# Autodesk Inventor assembly: Assembly1
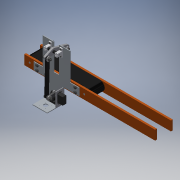
[picture p0: Inventor's stored thumbnail of the model, 180x180]
Saved by Autodesk Inventor 2019 (Build 230136000, 136)
## iProperties
Created: 2021-10-24
Part Number: Assembly1
Document SubType Name: Assembly
Designer: Mohamed Teleb
Sending System: Autodesk Inventor 2022
Preprocessor: ST-DEVELOPER v18.1
Title: C:\Users\Mohamed Teleb\OneDrive - Faculty of Engineering Ain Shams University\Documents\Inventor\AssemblyDesignOfMechatronics1\Assembly1.stp
Author: Mohamed Teleb
## Documents named in this file (32)
- C:\Users\Mohamed Teleb\OneDrive - Faculty of Engineering Ain Shams University\Desktop\DOM1STEP\Assembly1.iam
- C:\Users\Mohamed Teleb\OneDrive - Faculty of Engineering Ain Shams University\Desktop\DOM1STEP\Part1.ipt
- C:\Users\Mohamed Teleb\OneDrive - Faculty of Engineering Ain Shams University\Desktop\DOM1STEP\Part4.ipt
- C:\Users\Mohamed Teleb\OneDrive - Faculty of Engineering Ain Shams University\Desktop\DOM1STEP\Part7.ipt
- C:\Users\Mohamed Teleb\OneDrive - Faculty of Engineering Ain Shams University\Desktop\DOM1STEP\FilesFromInventor2019\SideToConveyer.ipt
- C:\Users\Mohamed Teleb\OneDrive - Faculty of Engineering Ain Shams University\Desktop\DOM1STEP\ISO 14583 - M8x25-4.8.ipt
- C:\Users\Mohamed Teleb\OneDrive - Faculty of Engineering Ain Shams University\Desktop\DOM1STEP\ISO 8738 - 8(2).ipt
- C:\Users\Mohamed Teleb\OneDrive - Faculty of Engineering Ain Shams University\Desktop\DOM1STEP\ISO 4034 - M8 - ISO.ipt
- C:\Users\Mohamed Teleb\OneDrive - Faculty of Engineering Ain Shams University\Desktop\DOM1STEP\StepperHolder.ipt
- C:\Users\Mohamed Teleb\OneDrive - Faculty of Engineering Ain Shams University\Desktop\DOM1STEP\FilesFromInventor2019\SK10.ipt
- C:\Users\Mohamed Teleb\OneDrive - Faculty of Engineering Ain Shams University\Desktop\DOM1STEP\ArmSupporterFinal.ipt
- C:\Users\Mohamed Teleb\OneDrive - Faculty of Engineering Ain Shams University\Desktop\DOM1STEP\Arm.ipt
- C:\Users\Mohamed Teleb\OneDrive - Faculty of Engineering Ain Shams University\Desktop\DOM1STEP\FilesFromInventor2019\Fixer.ipt
- C:\Users\Mohamed Teleb\OneDrive - Faculty of Engineering Ain Shams University\Desktop\DOM1STEP\FilesFromInventor2019\ConnectingRodtoTheArm.ipt
- C:\Users\Mohamed Teleb\OneDrive - Faculty of Engineering Ain Shams University\Desktop\DOM1STEP\FilesFromInventor2019\Cranck.ipt
- C:\Users\Mohamed Teleb\OneDrive - Faculty of Engineering Ain Shams University\Desktop\DOM1STEP\ServooHolderFinal.ipt
- C:\Users\Mohamed Teleb\OneDrive - Faculty of Engineering Ain Shams University\Desktop\DOM1STEP\FilesFromInventor2019\FeeTech FS5109M Metal Gear Servo Outer volume.ipt
- C:\Users\Mohamed Teleb\OneDrive - Faculty of Engineering Ain Shams University\Desktop\DOM1STEP\FilesFromInventor2019\CranckCouplerFromServo.ipt
- C:\Users\Mohamed Teleb\OneDrive - Faculty of Engineering Ain Shams University\Desktop\DOM1STEP\FilesFromInventor2019\Bearings.ipt
- C:\Users\Mohamed Teleb\OneDrive - Faculty of Engineering Ain Shams University\Desktop\DOM1STEP\FilesFromInventor2019\SuctionHolder.ipt
- C:\Users\Mohamed Teleb\OneDrive - Faculty of Engineering Ain Shams University\Desktop\DOM1STEP\ISO 7045 - M4 x 8_ - 4.8 - H - ISO.ipt
- C:\Users\Mohamed Teleb\OneDrive - Faculty of Engineering Ain Shams University\Desktop\DOM1STEP\ISO 7045 - M5 x 20_ - 4.8 - H - ISO.ipt
- C:\Users\Mohamed Teleb\OneDrive - Faculty of Engineering Ain Shams University\Desktop\DOM1STEP\ISO 7045 - M6 x 30_ - 4.8 - H - ISO.ipt
- C:\Users\Mohamed Teleb\OneDrive - Faculty of Engineering Ain Shams University\Desktop\DOM1STEP\ISO 7092 - ST 6 - 140 HV.ipt
- C:\Users\Mohamed Teleb\OneDrive - Faculty of Engineering Ain Shams University\Desktop\DOM1STEP\ISO 4034 - M6 - ISO.ipt
- C:\Users\Mohamed Teleb\OneDrive - Faculty of Engineering Ain Shams University\Desktop\DOM1STEP\ISO 7045 - M8 x 35_ - 4.8 - H - ISO.ipt
- C:\Users\Mohamed Teleb\OneDrive - Faculty of Engineering Ain Shams University\Desktop\DOM1STEP\ISO 7093 A - ST 8 - 140 HV.ipt
- C:\Users\Mohamed Teleb\OneDrive - Faculty of Engineering Ain Shams University\Desktop\DOM1STEP\ISO 4033 - M8 - ISO.ipt
- C:\Users\Mohamed Teleb\OneDrive - Faculty of Engineering Ain Shams University\Desktop\DOM1STEP\ISO 7045 - M2 x 16_ - 4.8 - H - ISO.ipt
- C:\Users\Mohamed Teleb\OneDrive - Faculty of Engineering Ain Shams University\Desktop\DOM1STEP\Supporterrrre.ipt
- C:\Users\Mohamed Teleb\OneDrive - Faculty of Engineering Ain Shams University\Desktop\DOM1STEP\ISO 7045 - M6 x 12_ - 4.8 - H - ISO.ipt
- C:\Users\Mohamed Teleb\OneDrive - Faculty of Engineering Ain Shams University\Desktop\DOM1STEP\ISO 7045 - M6 x 10_ - 4.8 - H - ISO.ipt
## Components (56 placed, 31 different names)
1. Part1:1 — Flush:2, Flush:4, Mate:4
2. Part4:1 — Mate:1, Flush:1, Flush:2
3. Part7:1 — Mate:3, Mate:4, Angle:1
4. Part1:2 — Mate:1, Flush:1, Mate:2, Flush:3, Mate:10, Mate:12, Mate:13, Mate:14
5. Part4:2 — Mate:2, Flush:3, Flush:4, Mate:3
6. SideToConveyer:3 — Mate:5, Mate:7, Mate:8, Mate:9, Mate:11, Mate:12, Mate:13, Mate:14, Mate:15, Mate:16, Mate:17, Mate:18, Mate:19, Mate:20, Mate:21, Mate:26, Mate:27, Mate:28, Mate:29, Mate:59, Mate:60, Mate:61, Mate:62, Mate:63, Mate:64
7. Screw ISO 14583:2011(E) M8x25-4.8:5 — Mate:10, Mate:11
8. ISO 8738 8:5
9. ISO 4034 M8:9
10. Screw ISO 14583:2011(E) M8x25-4.8:6 — Mate:15, Mate:16
11. Screw ISO 14583:2011(E) M8x25-4.8:7 — Mate:19, Mate:20
12. Screw ISO 14583:2011(E) M8x25-4.8:8 — Mate:17, Mate:18
13. ISO 8738 8:6
14. ISO 8738 8:7
15. ISO 8738 8:8
16. ISO 4034 M8:10
17. ISO 4034 M8:11
18. ISO 4034 M8:12
19. StepperHolder:2 — Mate:6, Mate:7, Mate:8, Mate:9, Mate:22, Mate:23, Mate:24, Mate:25, Mate:30, Flush:5, Mate:31
20. SK10:1 — Mate:62, Mate:63, Mate:64, Mate:65, Mate:67, Mate:69, Rotational:4, Rotational:5
21. SK10:2 — Mate:59, Mate:60, Mate:61, Mate:66, Rotational:2, Rotational:3
22. ArmSupporterFinal:1 — Mate:65, Mate:66, Mate:67, Mate:68, Mate:70, Mate:72
23. Arm:1 — Mate:70, Mate:71, Mate:73, Mate:74, Mate:79, Mate:80, Mate:88, Flush:6, Mate:89
24. Fixer:1 — Mate:72, Mate:73
25. Fixer:2 — Mate:68, Mate:69, Mate:71
26. ConnectingRodtoTheArm:1 — Mate:55, Mate:56, Mate:57, Mate:58, Mate:74, Mate:77, Mate:78
27. Cranck:1 — Mate:43, Mate:44, Mate:45, Mate:51, Mate:52, Mate:55, Mate:56
28. ServooHolderFinal:1 — Mate:30, Flush:5, Mate:31, Mate:32, Mate:33, Mate:34
29. FeeTech FS5109M Metal Gear Servo Outer volume:1 — Mate:32, Mate:33, Mate:34, Mate:35, Mate:36, Mate:37, Mate:38, Mate:39, Mate:40, Mate:41, Mate:42, Rotational:1
30. CranckCouplerFromServo:1 — Rotational:1, Mate:43, Mate:44, Mate:45, Mate:46, Mate:47, Mate:48, Mate:49, Mate:50
31. Bearings:1 — Mate:87, Mate:88, Flush:6
32. SuctionHolder:1 — Mate:83, Mate:84, Mate:85, Mate:86, Mate:89, Angle:1
33. ISO 7045 H M4 x 8 - 4.8 - H:1 — Mate:41, Mate:42
34. ISO 7045 H M4 x 8 - 4.8 - H:2 — Mate:35, Mate:36
35. ISO 7045 H M4 x 8 - 4.8 - H:3 — Mate:39, Mate:40
36. ISO 7045 H M4 x 8 - 4.8 - H:4 — Mate:37, Mate:38
37. ISO 7045 H M5 x 20 - 4.8 - H:1 — Rotational:5
38. ISO 7045 H M5 x 20 - 4.8 - H:2 — Rotational:4
39. ISO 7045 H M5 x 20 - 4.8 - H:3 — Rotational:3
40. ISO 7045 H M5 x 20 - 4.8 - H:4 — Rotational:2
41. ISO 7045 H M6 x 30 - 4.8 - H:1 — Mate:85, Mate:86, Mate:87
42. ISO 7092 ST 6 - 140 HV:1 — Mate:81, Mate:82, Mate:83, Mate:84
43. ISO 4034 M6:1 — Mate:81, Mate:82
44. ISO 7045 H M8 x 35 - 4.8 - H:1 — Mate:79, Mate:80
45. ISO 7093 A ST 8 - 140 HV - A:1 — Mate:75, Mate:76, Mate:77, Mate:78
46. ISO 4033 M8:1 — Mate:75, Mate:76
47. ISO 7045 H M8 x 35 - 4.8 - H:2 — Mate:57, Mate:58
48. ISO 7093 A ST 8 - 140 HV - A:2 — Mate:51, Mate:52, Mate:53, Mate:54
49. ISO 4034 M8:13 — Mate:53, Mate:54
50. ISO 7045 H M2 x 16 - 4.8 - H:2 — Mate:48, Mate:49, Mate:50
51. ISO 7045 H M2 x 16 - 4.8 - H:4 — Mate:46, Mate:47
52. Supporterrrree:1 — Mate:5, Mate:6, Mate:21
53. ISO 7045 H M6 x 12 - 4.8 - H:1 — Mate:26, Mate:27
54. ISO 7045 H M6 x 12 - 4.8 - H:2 — Mate:28, Mate:29
55. ISO 7045 H M6 x 10 - 4.8 - H:1 — Mate:22, Mate:23
56. ISO 7045 H M6 x 10 - 4.8 - H:2 — Mate:24, Mate:25
## Relationships (101: Mate 89, Flush 6, RevoluteJoint 5, Angle 1)
- Mate:1: Part4:1 ↔ Part1:2
- Flush:1: Part4:1 ↔ Part1:2
- Flush:2: Part1:1 ↔ Part4:1
- Mate:2: Part1:2 ↔ Part4:2
- Flush:3: Part1:2 ↔ Part4:2
- Flush:4: Part1:1 ↔ Part4:2
- Mate:3: Part7:1 ↔ Part4:2
- Mate:4 (1.5 mm): Part1:1 ↔ Part7:1
- Mate:5: SideToConveyer:3 ↔ Supporterrrree:1
- Mate:6: StepperHolder:2 ↔ Supporterrrree:1
- Mate:7: SideToConveyer:3 ↔ StepperHolder:2
- Mate:8: SideToConveyer:3 ↔ StepperHolder:2
- Mate:9: SideToConveyer:3 ↔ StepperHolder:2
- Mate:10: Part1:2 ↔ Screw ISO 14583:2011(E) M8x25-4.8:5
- Mate:11: SideToConveyer:3 ↔ Screw ISO 14583:2011(E) M8x25-4.8:5
- Mate:12: Part1:2 ↔ SideToConveyer:3
- Mate:13: Part1:2 ↔ SideToConveyer:3
- Mate:14: Part1:2 ↔ SideToConveyer:3
- Mate:15: SideToConveyer:3 ↔ Screw ISO 14583:2011(E) M8x25-4.8:6
- Mate:16: SideToConveyer:3 ↔ Screw ISO 14583:2011(E) M8x25-4.8:6
- Mate:17: SideToConveyer:3 ↔ Screw ISO 14583:2011(E) M8x25-4.8:8
- Mate:18: SideToConveyer:3 ↔ Screw ISO 14583:2011(E) M8x25-4.8:8
- Mate:19: SideToConveyer:3 ↔ Screw ISO 14583:2011(E) M8x25-4.8:7
- Mate:20: SideToConveyer:3 ↔ Screw ISO 14583:2011(E) M8x25-4.8:7
- Mate:21: SideToConveyer:3 ↔ Supporterrrree:1
- Mate:22: StepperHolder:2 ↔ ISO 7045 H M6 x 10 - 4.8 - H:1
- Mate:23: StepperHolder:2 ↔ ISO 7045 H M6 x 10 - 4.8 - H:1
- Mate:24: StepperHolder:2 ↔ ISO 7045 H M6 x 10 - 4.8 - H:2
- Mate:25: StepperHolder:2 ↔ ISO 7045 H M6 x 10 - 4.8 - H:2
- Mate:26: SideToConveyer:3 ↔ ISO 7045 H M6 x 12 - 4.8 - H:1
- Mate:27: SideToConveyer:3 ↔ ISO 7045 H M6 x 12 - 4.8 - H:1
- Mate:28: SideToConveyer:3 ↔ ISO 7045 H M6 x 12 - 4.8 - H:2
- Mate:29: SideToConveyer:3 ↔ ISO 7045 H M6 x 12 - 4.8 - H:2
- Mate:30: StepperHolder:2 ↔ ServooHolderFinal:1
- Flush:5: StepperHolder:2 ↔ ServooHolderFinal:1
- Mate:31: StepperHolder:2 ↔ ServooHolderFinal:1
- Mate:32: ServooHolderFinal:1 ↔ FeeTech FS5109M Metal Gear Servo Outer volume:1
- Mate:33: ServooHolderFinal:1 ↔ FeeTech FS5109M Metal Gear Servo Outer volume:1
- Mate:34: ServooHolderFinal:1 ↔ FeeTech FS5109M Metal Gear Servo Outer volume:1
- Mate:35: FeeTech FS5109M Metal Gear Servo Outer volume:1 ↔ ISO 7045 H M4 x 8 - 4.8 - H:2
- Mate:36: FeeTech FS5109M Metal Gear Servo Outer volume:1 ↔ ISO 7045 H M4 x 8 - 4.8 - H:2
- Mate:37: FeeTech FS5109M Metal Gear Servo Outer volume:1 ↔ ISO 7045 H M4 x 8 - 4.8 - H:4
- Mate:38: FeeTech FS5109M Metal Gear Servo Outer volume:1 ↔ ISO 7045 H M4 x 8 - 4.8 - H:4
- Mate:39: FeeTech FS5109M Metal Gear Servo Outer volume:1 ↔ ISO 7045 H M4 x 8 - 4.8 - H:3
- Mate:40: FeeTech FS5109M Metal Gear Servo Outer volume:1 ↔ ISO 7045 H M4 x 8 - 4.8 - H:3
- Mate:41: FeeTech FS5109M Metal Gear Servo Outer volume:1 ↔ ISO 7045 H M4 x 8 - 4.8 - H:1
- Mate:42: FeeTech FS5109M Metal Gear Servo Outer volume:1 ↔ ISO 7045 H M4 x 8 - 4.8 - H:1
- Rotational:1 [RevoluteJoint] (0.4 mm): FeeTech FS5109M Metal Gear Servo Outer volume:1 ↔ CranckCouplerFromServo:1
- Mate:43: Cranck:1 ↔ CranckCouplerFromServo:1
- Mate:44: Cranck:1 ↔ CranckCouplerFromServo:1
- Mate:45: Cranck:1 ↔ CranckCouplerFromServo:1
- Mate:46: CranckCouplerFromServo:1 ↔ ISO 7045 H M2 x 16 - 4.8 - H:4
- Mate:47: CranckCouplerFromServo:1 ↔ ISO 7045 H M2 x 16 - 4.8 - H:4
- Mate:48: CranckCouplerFromServo:1 ↔ ISO 7045 H M2 x 16 - 4.8 - H:2
- Mate:49: CranckCouplerFromServo:1 ↔ ISO 7045 H M2 x 16 - 4.8 - H:2
- Mate:50: CranckCouplerFromServo:1 ↔ ISO 7045 H M2 x 16 - 4.8 - H:2
- Mate:51: Cranck:1 ↔ ISO 7093 A ST 8 - 140 HV - A:2
- Mate:52: Cranck:1 ↔ ISO 7093 A ST 8 - 140 HV - A:2
- Mate:53: ISO 7093 A ST 8 - 140 HV - A:2 ↔ ISO 4034 M8:13
- Mate:54: ISO 7093 A ST 8 - 140 HV - A:2 ↔ ISO 4034 M8:13
- Mate:55: ConnectingRodtoTheArm:1 ↔ Cranck:1
- Mate:56: ConnectingRodtoTheArm:1 ↔ Cranck:1
- Mate:57: ConnectingRodtoTheArm:1 ↔ ISO 7045 H M8 x 35 - 4.8 - H:2
- Mate:58: ConnectingRodtoTheArm:1 ↔ ISO 7045 H M8 x 35 - 4.8 - H:2
- Mate:59: SideToConveyer:3 ↔ SK10:2
- Mate:60: SideToConveyer:3 ↔ SK10:2
- Mate:61: SideToConveyer:3 ↔ SK10:2
- Mate:62: SideToConveyer:3 ↔ SK10:1
- Mate:63: SideToConveyer:3 ↔ SK10:1
- Mate:64: SideToConveyer:3 ↔ SK10:1
- Mate:65: SK10:1 ↔ ArmSupporterFinal:1
- Mate:66: SK10:2 ↔ ArmSupporterFinal:1
- Mate:67: SK10:1 ↔ ArmSupporterFinal:1
- Mate:68: ArmSupporterFinal:1 ↔ Fixer:2
- Mate:69: SK10:1 ↔ Fixer:2
- Mate:70: ArmSupporterFinal:1 ↔ Arm:1
- Mate:71: Arm:1 ↔ Fixer:2
- Mate:72: ArmSupporterFinal:1 ↔ Fixer:1
- Mate:73: Arm:1 ↔ Fixer:1
- Mate:74: Arm:1 ↔ ConnectingRodtoTheArm:1
- Mate:75: ISO 7093 A ST 8 - 140 HV - A:1 ↔ ISO 4033 M8:1
- Mate:76: ISO 7093 A ST 8 - 140 HV - A:1 ↔ ISO 4033 M8:1
- Mate:77: ConnectingRodtoTheArm:1 ↔ ISO 7093 A ST 8 - 140 HV - A:1
- Mate:78: ConnectingRodtoTheArm:1 ↔ ISO 7093 A ST 8 - 140 HV - A:1
- Mate:79: Arm:1 ↔ ISO 7045 H M8 x 35 - 4.8 - H:1
- Mate:80: Arm:1 ↔ ISO 7045 H M8 x 35 - 4.8 - H:1
- Mate:81: ISO 7092 ST 6 - 140 HV:1 ↔ ISO 4034 M6:1
- Mate:82: ISO 7092 ST 6 - 140 HV:1 ↔ ISO 4034 M6:1
- Mate:83: SuctionHolder:1 ↔ ISO 7092 ST 6 - 140 HV:1
- Mate:84: SuctionHolder:1 ↔ ISO 7092 ST 6 - 140 HV:1
- Mate:85: SuctionHolder:1 ↔ ISO 7045 H M6 x 30 - 4.8 - H:1
- Mate:86: SuctionHolder:1 ↔ ISO 7045 H M6 x 30 - 4.8 - H:1
- Mate:87: Bearings:1 ↔ ISO 7045 H M6 x 30 - 4.8 - H:1
- Mate:88: Arm:1 ↔ Bearings:1
- Flush:6 (1 mm): Arm:1 ↔ Bearings:1
- Mate:89 (0.75 mm): Arm:1 ↔ SuctionHolder:1
- Rotational:2 [RevoluteJoint]: SK10:2 ↔ ISO 7045 H M5 x 20 - 4.8 - H:4
- Rotational:3 [RevoluteJoint]: SK10:2 ↔ ISO 7045 H M5 x 20 - 4.8 - H:3
- Rotational:4 [RevoluteJoint]: SK10:1 ↔ ISO 7045 H M5 x 20 - 4.8 - H:2
- Rotational:5 [RevoluteJoint]: SK10:1 ↔ ISO 7045 H M5 x 20 - 4.8 - H:1
- Angle:1 (179.9087 deg): Part7:1 ↔ SuctionHolder:1
